# Autodesk Inventor assembly: ASY NDM-VOS_powder_hopper
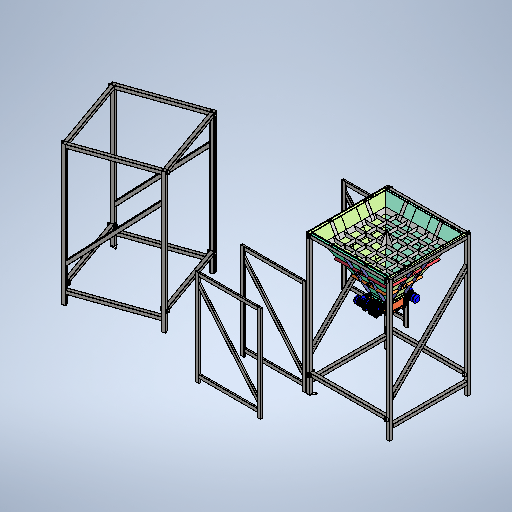
[picture p0: Inventor's stored thumbnail of the model, 512x512]
Saved by Autodesk Inventor 2025.1 (Build 291241020, 241B)
## iProperties
Created: 2024-07-24
Part Number: ASY NDM-VOS_powder_hopper
Document SubType Name: Assembly
Designer: admin
Author: admin
## Documents named in this file (19)
- C:\Users\user\YandexDisk-badmisterfox\домашниий пк\Inventor\NDM-VOS_powder_hopper\ASY NDM-VOS_powder_hopper.iam
- C:\Users\user\YandexDisk-badmisterfox\домашниий пк\Inventor\NDM-VOS_powder_hopper\human 01\ч ASY human dummy 01.iam
- C:\Users\user\YandexDisk-badmisterfox\домашниий пк\Inventor\NDM-VOS_powder_hopper\NDM-VOS dummy3.ipt
- C:\Users\user\YandexDisk-badmisterfox\домашниий пк\Inventor\NDM-VOS_powder_hopper\NDM-VOS dummy5.ipt
- C:\Users\user\YandexDisk-badmisterfox\домашниий пк\Inventor\NDM-VOS_powder_hopper\NDM-VOS dummy FLOOR.ipt
- C:\Users\user\YandexDisk-badmisterfox\домашниий пк\Inventor\NDM-VOS_powder_hopper\NDM-VOS dummy Crane.ipt
- C:\Users\user\YandexDisk-badmisterfox\домашниий пк\Inventor\NDM-VOS_powder_hopper\NDM-VOS dummy upstairse.ipt
- C:\Users\user\YandexDisk-badmisterfox\домашниий пк\Inventor\NDM-VOS_powder_hopper\Workspaces\Workspace\Cone\ASY MSC 100 cone.iam
- C:\Users\user\YandexDisk-badmisterfox\домашниий пк\Inventor\NDM-VOS_powder_hopper\ASY HPR 200  Frame.iam
- C:\Users\user\YandexDisk-badmisterfox\домашниий пк\Inventor\NDM-VOS_powder_hopper\TM06198C pump.ipt
- C:\Users\user\YandexDisk-badmisterfox\домашниий пк\Inventor\NDM-VOS_powder_hopper\ASY HPR 300 Frame human.iam
- C:\Users\user\YandexDisk-badmisterfox\домашниий пк\Inventor\NDM-VOS_powder_hopper\ASY_Ступень.iam
- C:\Users\user\YandexDisk-badmisterfox\домашниий пк\Inventor\NDM-VOS_powder_hopper\ASY стойка.iam
- C:\Users\user\YandexDisk-badmisterfox\домашниий пк\Inventor\NDM-VOS_powder_hopper\ISO 4019 - 80x40x2 - 2500.ipt
- C:\Users\user\YandexDisk-badmisterfox\домашниий пк\Inventor\NDM-VOS_powder_hopper\ASY NVPH-400 shredder.iam
- C:\Users\user\YandexDisk-badmisterfox\домашниий пк\Inventor\Content Center Files\en-US\ISO 4775\ISO 4775 - M12.ipt
- C:\Users\user\YandexDisk-badmisterfox\домашниий пк\Inventor\NDM-VOS_powder_hopper\3d party\PCRV080-075SHFA_MS80B5\PCRV080-075SHFA_MS80B5\PCRV080-075SHFA_MS80B5.ipt
- C:\Users\user\YandexDisk-badmisterfox\домашниий пк\Inventor\NDM-VOS_powder_hopper\ASY NVPH-300 hopper.iam
- C:\Users\user\YandexDisk-badmisterfox\домашниий пк\Inventor\NDM-VOS_powder_hopper\ASY Augur motor frame 500.iam
## Components (40 placed, 18 different names)
1. NDM-VOS dummy3:2 — Mate:6, Mate:8, Mate:9, Flush:15
2. NDM-VOS dummy5:1 — Mate:14, Flush:16
3. NDM-VOS dummy5:2 — Flush:9, Flush:15, Mate:14
4. ч ASY human dummy 01:1 [sub-assembly]
5. NDM-VOS dummy FLOOR:1 — Mate:5, Mate:6, Mate:8, Mate:10, Flush:16, Mate:18
6. NDM-VOS dummy Crane:1 — Mate:10
7. NDM-VOS dummy upstairse:1 — Mate:18, Mate:23
8. ASY MSC 100 CONE:1 [sub-assembly] — Mate:20, Rigid:27
9. ASY HPR 200  Frame:1 [sub-assembly] — Mate:20, Mate:35, Rigid:31
10. TM06198C pump:1
11. ASY HPR 300 Frame human:1 [sub-assembly]
12. ASY HPR 200  Frame:2 [sub-assembly]
13. ASY стойка:1 [sub-assembly] — Rigid:5, Rigid:6, Mate:35
14. ASY стойка:2 [sub-assembly] — Rigid:4, Rigid:31
15. ASY стойка:3 [sub-assembly] — Rigid:4, Flush:25
16. ISO 4019 - 80x40x2 - 2700:1 — Rigid:5
17. ISO 4019 - 80x40x2 - 2700:2
18. ISO 4019 - 80x40x2 - 2700:3 — Rigid:6, Flush:24, Mate:24
19. ASY MSC 100 CONE:2 [sub-assembly] — Rigid:29
20. TM06198C pump:2
21. ASY NVPH-400 shredder:1 [sub-assembly] — Rigid:27, Mate:31, Mate:32
22. ISO 4775 M12:1 — Mate:31, Mate:32
23. PCRV080-075SHFA_MS80B5:1
24. ASY NVPH-300 hopper:1 [sub-assembly]
25. ASY NVPH-400 shredder:2 [sub-assembly] — Rigid:29, Rigid:30
26. ASY NVPH-300 hopper:2 [sub-assembly] — Rigid:30
27. NDM-VOS dummy3:1 — Mate:5, Mate:9
28. ASY Augur motor frame 500:1 [sub-assembly]
29. ASY_Ступень:1 [sub-assembly] — Flush:24, Mate:23, Mate:24, Flush:25
30. ASY_Ступень:2 [sub-assembly]
31. ASY_Ступень:3 [sub-assembly]
32. ASY_Ступень:4 [sub-assembly]
33. ASY_Ступень:5 [sub-assembly]
34. ASY_Ступень:6 [sub-assembly]
35. ASY_Ступень:7 [sub-assembly]
36. ASY_Ступень:8 [sub-assembly]
37. ASY_Ступень:9 [sub-assembly]
38. ASY_Ступень:10 [sub-assembly]
39. ASY_Ступень:11 [sub-assembly]
40. ASY_Ступень:12 [sub-assembly]
## Component patterns: (12 elements, first: ASY_Ступень:1)
## Relationships (35: Mate 17, Flush 9, WeldJoint 8, RevoluteJoint 1)
- Flush:9: NDM-VOS dummy5:2
- Mate:5: NDM-VOS dummy FLOOR:1 ↔ NDM-VOS dummy3:1
- Mate:6: NDM-VOS dummy3:2 ↔ NDM-VOS dummy FLOOR:1
- Mate:8 (1200 mm): NDM-VOS dummy3:2 ↔ NDM-VOS dummy FLOOR:1
- Mate:9 (-1830 mm): NDM-VOS dummy3:2 ↔ NDM-VOS dummy3:1
- Mate:10 (3500 mm): NDM-VOS dummy FLOOR:1 ↔ NDM-VOS dummy Crane:1
- [Mate]: NDM-VOS dummy3:2 ↔ ASY MSC 100 CONE:1
- Flush:15: NDM-VOS dummy3:2 ↔ NDM-VOS dummy5:2
- Mate:14: NDM-VOS dummy5:1 ↔ NDM-VOS dummy5:2
- Flush:16: NDM-VOS dummy5:1 ↔ NDM-VOS dummy FLOOR:1
- Mate:18: NDM-VOS dummy FLOOR:1 ↔ NDM-VOS dummy upstairse:1
- [Flush]: ASY HPR 200  Frame:1
- Mate:20: ASY MSC 100 CONE:1 ↔ ASY HPR 200  Frame:1
- Rigid:4 [WeldJoint] (1000 mm): ASY стойка:2 ↔ ASY стойка:3
- Rigid:5 [WeldJoint]: ASY стойка:1 ↔ ISO 4019 - 80x40x2 - 2700:1
- Rigid:6 [WeldJoint]: ASY стойка:1 ↔ ISO 4019 - 80x40x2 - 2700:3
- Flush:24 (182 mm): ISO 4019 - 80x40x2 - 2700:3 ↔ ASY_Ступень:1
- Mate:23: NDM-VOS dummy upstairse:1 ↔ ASY_Ступень:1
- Mate:24: ISO 4019 - 80x40x2 - 2700:3 ↔ ASY_Ступень:1
- Flush:25: ASY стойка:3 ↔ ASY_Ступень:1
- Rigid:27 [WeldJoint]: ASY MSC 100 CONE:1 ↔ ASY NVPH-400 shredder:1
- [WeldJoint]: ASY NVPH-400 shredder:1 ↔ ASY NVPH-300 hopper:1
- [Mate]: ASY NVPH-400 shredder:1 ↔ ASY NVPH-300 hopper:1
- [Flush]: ASY NVPH-400 shredder:1 ↔ ASY NVPH-300 hopper:1
- Mate:31: ASY NVPH-400 shredder:1 ↔ ISO 4775 M12:1
- Mate:32: ASY NVPH-400 shredder:1 ↔ ISO 4775 M12:1
- [RevoluteJoint] (100 mm): PCRV080-075SHFA_MS80B5:1 ↔ ASY NVPH-300 hopper:1
- [Mate]: ASY NVPH-400 shredder:1 ↔ ASY NVPH-300 hopper:1
- Rigid:29 [WeldJoint]: ASY MSC 100 CONE:2 ↔ ASY NVPH-400 shredder:2
- Rigid:30 [WeldJoint]: ASY NVPH-400 shredder:2 ↔ ASY NVPH-300 hopper:2
- [Flush]: NDM-VOS dummy3:1 ↔ ASY Augur motor frame 500:1
- [Mate]: NDM-VOS dummy3:1 ↔ ASY Augur motor frame 500:1
- [Flush]: NDM-VOS dummy3:1 ↔ ASY Augur motor frame 500:1
- Mate:35: ASY HPR 200  Frame:1 ↔ ASY стойка:1
- Rigid:31 [WeldJoint]: ASY HPR 200  Frame:1 ↔ ASY стойка:2
